# Autodesk Inventor assembly: gyroGearHeadAssembly06
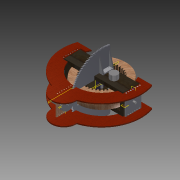
[picture p0: Inventor's stored thumbnail of the model, 180x180]
Saved by Autodesk Inventor 2013 (Build 170138000, 138)
## iProperties
Created: 2013-02-24
Part Number: gyroGearHeadAssembly06
Document SubType Name: Assembly
Designer: Nano
Author: Nano
## Documents named in this file (22)
- C:\Users\Nano\Documents\InventorByron\InventorMasterProject\gyroPhone01\gyroGearHeadAssembly06.iam
- C:\Users\Nano\Documents\InventorByron\InventorMasterProject\gyroPhone01\littleGear01.ipt
- C:\Users\Nano\Documents\InventorByron\InventorMasterProject\gyroPhone01\gearGuideRings.ipt
- C:\Users\Nano\Documents\InventorByron\InventorMasterProject\gyroPhone01\bigGearSection01.ipt
- C:\Users\Nano\Documents\InventorByron\InventorMasterProject\gyroPhone01\brace01.ipt
- C:\Users\Nano\Documents\InventorByron\InventorMasterProject\gyroPhone01\brace01_MIR1.ipt
- C:\Users\Nano\Documents\InventorByron\InventorMasterProject\gyroPhone01\brace02_MIR.ipt
- C:\Users\Nano\Documents\InventorByron\InventorMasterProject\gyroPhone01\basePlate01.ipt
- C:\Users\Nano\Documents\InventorByron\InventorMasterProject\gyroPhone01\basePlate01_MIR2.ipt
- C:\Users\Nano\Documents\InventorByron\InventorMasterProject\gyroPhone01\basePlate01_MIR3.ipt
- C:\Users\Nano\Documents\InventorByron\InventorMasterProject\gyroPhone01\basePlate01_MIR2_MIR.ipt
- C:\Users\Nano\Documents\InventorByron\InventorMasterProject\gyroPhone01\gyroWheelCradle01.ipt
- C:\Users\Nano\Documents\InventorByron\InventorMasterProject\gyroPhone01\shortEndAxel.ipt
- C:\Users\Nano\Documents\InventorByron\InventorMasterProject\gyroPhone01\shortEndAxel_MIR.ipt
- C:\Users\Nano\Documents\InventorByron\InventorMasterProject\gyroPhone01\wheelAxel01.ipt
- C:\Users\Nano\Documents\InventorByron\InventorMasterProject\gyroPhone01\motorWheelAssembly01.iam
- C:\Users\Nano\Documents\InventorByron\InventorMasterProject\gyroPhone01\gyroYoke01.ipt
- C:\Users\Nano\Documents\InventorByron\InventorMasterProject\gyroPhone01\yokeEndBlock.ipt
- C:\Users\Nano\Documents\InventorByron\InventorMasterProject\gyroPhone01\stepperShaftCollar.ipt
- C:\Users\Nano\Documents\InventorByron\InventorMasterProject\gyroPhone01\stepperMotorBodyPlusAxel.iam
- C:\Users\Nano\Documents\InventorByron\InventorMasterProject\gyroPhone01\gyroYoke01_MIR1.ipt
- C:\Users\Nano\Documents\InventorByron\InventorMasterProject\gyroPhone01\gearAssemblyTake02\stepperMotorMountPlate01resized01.ipt
## Components (23 placed, 21 different names)
1. Spur Gear1:1 — Mate:3, Mate:5, Mate:6, Mate:7, gearsFlushWithEachOther, Mate:31, Mate:36
2. gearGuideRings:1 — Mate:3, Mate:6
3. gearGuideRings:2 — Mate:5, Mate:7, Mate:30
4. Spur Gear2:1 — gearsFlushWithEachOther, Angle:1, Flush:3, Mate:10, Mate:11, Mate:12, Mate:13, Mate:14, Flush:4, Mate:16, Mate:17, Mate:18, Mate:19
5. brace01:1 — Flush:3, Mate:10, Mate:11, Mate:15
6. brace01_MIR1:1
7. brace02_MIR:1 — Mate:12, Mate:13, Mate:16
8. basePlate01:1 — Mate:14, Flush:4, Mate:15
9. basePlate01_MIR2:1
10. basePlate01_MIR3:1
11. basePlate01_MIR2_MIR:1
12. gyroWheelCradle01:1 — Mate:17, Mate:18, Mate:19, Mate:20, Flush:5, Mate:21, Flush:6, Mate:23, Flush:7, Mate:24, Mate:25
13. shortEndAxel:1 — Mate:20, Flush:5, Angle:2
14. shortEndAxel_MIR:1 — Mate:34
15. wheelAxel01:1 — Mate:21, Flush:6, Mate:22
16. motorWheelAssembly01:1 [sub-assembly] — Mate:22, Mate:23, Angle:2
17. gyroYoke01:1 — Flush:7, Mate:24, Mate:25, Flush:8, Mate:26, Mate:27, Mate:35, Mate:9, Flush:9, Mate:36
18. yokeEndBlock:1 — Flush:8, Mate:26, Mate:27
19. stepperShaftCollar:1 — Mate:30
20. stepperMotorMountPlate01resized01:1 — Angle:1, Mate:32, Mate:33
21. stepperMotorBodyPlusAxel:1 [sub-assembly] — Mate:31, Mate:32, Mate:33
22. gyroYoke01_MIR1:1 — Flush:9
23. yokeEndBlock:2 — Mate:34, Mate:35, Mate:9
## Relationships (40: Mate 30, Flush 8, Angle 2)
- Mate:3: Spur Gear1:1 ↔ gearGuideRings:1
- Mate:5: Spur Gear1:1 ↔ gearGuideRings:2
- Mate:6: Spur Gear1:1 ↔ gearGuideRings:1
- Mate:7: Spur Gear1:1 ↔ gearGuideRings:2
- gearsFlushWithEachOther [Flush]: Spur Gear1:1 ↔ Spur Gear2:1
- Angle:1 (0 deg): Spur Gear2:1 ↔ stepperMotorMountPlate01resized01:1
- Flush:3: Spur Gear2:1 ↔ brace01:1
- Mate:10: Spur Gear2:1 ↔ brace01:1
- Mate:11: Spur Gear2:1 ↔ brace01:1
- Mate:12: Spur Gear2:1 ↔ brace02_MIR:1
- Mate:13: Spur Gear2:1 ↔ brace02_MIR:1
- Mate:14: Spur Gear2:1 ↔ basePlate01:1
- Flush:4: Spur Gear2:1 ↔ basePlate01:1
- Mate:15: brace01:1 ↔ basePlate01:1
- Mate:16: Spur Gear2:1 ↔ brace02_MIR:1
- Mate:17: Spur Gear2:1 ↔ gyroWheelCradle01:1
- Mate:18: Spur Gear2:1 ↔ gyroWheelCradle01:1
- Mate:19: Spur Gear2:1 ↔ gyroWheelCradle01:1
- Mate:20: gyroWheelCradle01:1 ↔ shortEndAxel:1
- Flush:5: gyroWheelCradle01:1 ↔ shortEndAxel:1
- Mate:21: gyroWheelCradle01:1 ↔ wheelAxel01:1
- Flush:6: gyroWheelCradle01:1 ↔ wheelAxel01:1
- Mate:22: wheelAxel01:1 ↔ motorWheelAssembly01:1
- Mate:23 (5.5626 mm): gyroWheelCradle01:1 ↔ motorWheelAssembly01:1
- Angle:2 (0 deg): shortEndAxel:1 ↔ motorWheelAssembly01:1
- Flush:7: gyroWheelCradle01:1 ↔ gyroYoke01:1
- Mate:24 (3.175 mm): gyroWheelCradle01:1 ↔ gyroYoke01:1
- Mate:25 (6.35 mm): gyroWheelCradle01:1 ↔ gyroYoke01:1
- Flush:8: gyroYoke01:1 ↔ yokeEndBlock:1
- Mate:26: gyroYoke01:1 ↔ yokeEndBlock:1
- Mate:27: gyroYoke01:1 ↔ yokeEndBlock:1
- Mate:30: gearGuideRings:2 ↔ stepperShaftCollar:1
- Mate:31: Spur Gear1:1 ↔ stepperMotorBodyPlusAxel:1
- Mate:32: stepperMotorMountPlate01resized01:1 ↔ stepperMotorBodyPlusAxel:1
- Mate:33: stepperMotorMountPlate01resized01:1 ↔ stepperMotorBodyPlusAxel:1
- Mate:34: shortEndAxel_MIR:1 ↔ yokeEndBlock:2
- Mate:35: gyroYoke01:1 ↔ yokeEndBlock:2
- Mate:9: gyroYoke01:1 ↔ yokeEndBlock:2
- Flush:9: gyroYoke01:1 ↔ gyroYoke01_MIR1:1
- Mate:36: Spur Gear1:1 ↔ gyroYoke01:1
